# Autodesk Inventor assembly: Assembly_Huawei_P20_Microscope
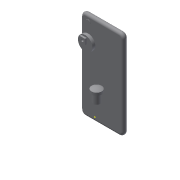
[picture p0: Inventor's stored thumbnail of the model, 180x180]
Saved by Autodesk Inventor 2019 (Build 230136000, 136)
## iProperties
Created: 2019-08-19
Part Number: Assembly_Huawei_P20_Microscope
Document SubType Name: Assembly
Designer: diederichbenedict
Author: diederichbenedict
## Documents named in this file (5)
- C:\Users\diederichbenedict\Dropbox\Dokumente\Promotion\PROJECTS\STORMoChip\INVENTOR\Nanoscopy-on-a-cheap\Assembly_Huawei_P20_Microscope.iam
- C:\Users\diederichbenedict\Dropbox\Dokumente\Promotion\PROJECTS\STORMoChip\INVENTOR\Nanoscopy-on-a-cheap\00_Huawei_P20.ipt
- C:\Users\diederichbenedict\Dropbox\Dokumente\Promotion\PROJECTS\STORMoChip\INVENTOR\Nanoscopy-on-a-cheap\100_CCTV_Fisheye_Starlight_f2.8mm_Fno_1.4.ipt
- C:\Users\diederichbenedict\Dropbox\Dokumente\Promotion\PROJECTS\STORMoChip\INVENTOR\Nanoscopy-on-a-cheap\100_chroma_HQ675_55.ipt
- C:\Users\diederichbenedict\Dropbox\Dokumente\Promotion\PROJECTS\STORMoChip\INVENTOR\Nanoscopy-on-a-cheap\00_Huawei_P20_Lens.ipt
## Components (4 placed, 4 different names)
1. 00_Huawei_P20:1 — Mate:1, Tangent:1, Tangent:2, Angle:1, Mate:3
2. 100_CCTV_Fisheye_Starlight_f2.8mm_Fno_1.4:1
3. 100_chroma_HQ675_55:1 — Mate:1, Tangent:1, Tangent:2, Mate:4
4. 00_Huawei_P20_Lens:1 — Angle:1, Mate:3, Mate:4
## Relationships (6: Mate 3, Tangent 2, Angle 1)
- Mate:1: 00_Huawei_P20:1 ↔ 100_chroma_HQ675_55:1
- Tangent:1: 00_Huawei_P20:1 ↔ 100_chroma_HQ675_55:1
- Tangent:2 (1 mm): 00_Huawei_P20:1 ↔ 100_chroma_HQ675_55:1
- Angle:1 (0 deg): 00_Huawei_P20:1 ↔ 00_Huawei_P20_Lens:1
- Mate:3: 00_Huawei_P20:1 ↔ 00_Huawei_P20_Lens:1
- Mate:4 (0.5 mm): 100_chroma_HQ675_55:1 ↔ 00_Huawei_P20_Lens:1
